# Autodesk Inventor assembly: Assembly1
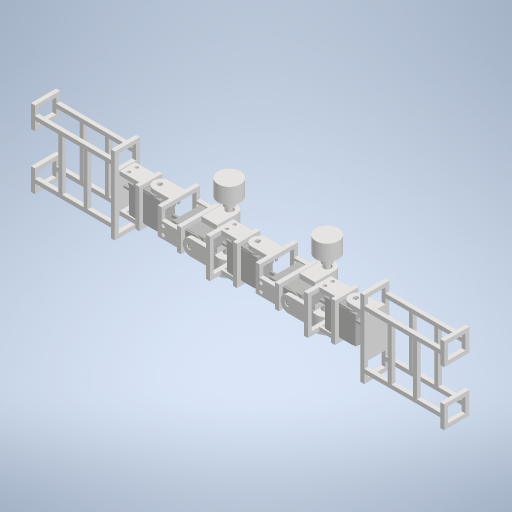
[picture p0: Inventor's stored thumbnail of the model, 512x512]
Saved by Autodesk Inventor 2024 (Build 280153000, 153)
## iProperties
Created: 2023-06-11
Part Number: Assembly1
Document SubType Name: Assembly
Designer: abhin
Author: abhin
## Documents named in this file (8)
- D:\Parth Folder\ES117\3D Model\Prototype 2\MBody(1).iam
- D:\Parth Folder\ES117\3D Model\Prototype 2\MG996R.ipt
- D:\Parth Folder\ES117\3D Model\Prototype 2\Sub Unit.ipt
- D:\Parth Folder\ES117\3D Model\Prototype 2\Wheel Holder.ipt
- D:\Parth Folder\ES117\3D Model\Prototype 2\Axis(1).ipt
- D:\Parth Folder\ES117\3D Model\Prototype 2\Small Wheels.ipt
- D:\Parth Folder\ES117\3D Model\Prototype 2\MHead(1).ipt
- D:\Parth Folder\ES117\3D Model\Prototype 2\MTail(1).ipt
## Components (19 placed, 7 different names)
1. MG996R:1 — Mate:1, Mate:2, Flush:1, Mate:31, Mate:32
2. Sub Unit:1 — Mate:1, Mate:2, Flush:1, Mate:3, Mate:4
3. MG996R:2 — Mate:3, Mate:4, Mate:5, Mate:6, Flush:2, Mate:19, Mate:20, Flush:6
4. Sub Unit:2 — Mate:5, Mate:6, Flush:2, Mate:9, Mate:10
5. MG996R:3 — Mate:9, Mate:10
6. Sub Unit:3 — Mate:13, Mate:14
7. MG996R:4 — Mate:13, Mate:14, Mate:17, Mate:18, Flush:5
8. Sub Unit:4 — Mate:15, Mate:16
9. MG996R:5 — Mate:15, Mate:16, Flush:9, Mate:33, Mate:34
10. Wheel Holder:1 — Mate:17, Mate:18, Flush:5, Mate:21, Flush:7
11. Wheel Holder:2 — Mate:19, Mate:20, Flush:6, Mate:22, Flush:8
12. Axis(1):1 — Mate:21, Flush:7, Mate:23, Mate:26, Mate:27, Mate:30
13. Axis(1):2 — Mate:22, Flush:8, Mate:24, Mate:25, Mate:28, Mate:29
14. Small Wheels:1 — Mate:26, Mate:30
15. Small Wheels:2 — Mate:25, Mate:29
16. Small Wheels:3 — Mate:23, Mate:27
17. Small Wheels:4 — Mate:24, Mate:28
18. MHead(1):1 — Mate:31, Mate:32
19. MTail(1):1 — Flush:9, Mate:33, Mate:34
## Relationships (43: Mate 34, Flush 9)
- Mate:1: MG996R:1 ↔ Sub Unit:1
- Mate:2: MG996R:1 ↔ Sub Unit:1
- Flush:1: MG996R:1 ↔ Sub Unit:1
- Mate:3: Sub Unit:1 ↔ MG996R:2
- Mate:4: Sub Unit:1 ↔ MG996R:2
- Mate:5: MG996R:2 ↔ Sub Unit:2
- Mate:6: MG996R:2 ↔ Sub Unit:2
- Flush:2: MG996R:2 ↔ Sub Unit:2
- [Mate]: MG996R:3 ↔ Sub Unit:3
- [Mate]: MG996R:3 ↔ Sub Unit:3
- [Flush]: MG996R:3 ↔ Sub Unit:3
- Mate:9: Sub Unit:2 ↔ MG996R:3
- Mate:10: Sub Unit:2 ↔ MG996R:3
- [Mate]: MG996R:4 ↔ Sub Unit:4
- [Mate]: MG996R:4 ↔ Sub Unit:4
- [Flush]: MG996R:4 ↔ Sub Unit:4
- Mate:13: Sub Unit:3 ↔ MG996R:4
- Mate:14: Sub Unit:3 ↔ MG996R:4
- Mate:15: Sub Unit:4 ↔ MG996R:5
- Mate:16: Sub Unit:4 ↔ MG996R:5
- Mate:17: MG996R:4 ↔ Wheel Holder:1
- Mate:18: MG996R:4 ↔ Wheel Holder:1
- Flush:5: MG996R:4 ↔ Wheel Holder:1
- Mate:19: MG996R:2 ↔ Wheel Holder:2
- Mate:20: MG996R:2 ↔ Wheel Holder:2
- Flush:6: MG996R:2 ↔ Wheel Holder:2
- Mate:21: Wheel Holder:1 ↔ Axis(1):1
- Mate:22: Wheel Holder:2 ↔ Axis(1):2
- Flush:7 (30 mm): Wheel Holder:1 ↔ Axis(1):1
- Flush:8 (30 mm): Wheel Holder:2 ↔ Axis(1):2
- Mate:23: Axis(1):1 ↔ Small Wheels:3
- Mate:24: Axis(1):2 ↔ Small Wheels:4
- Mate:25: Axis(1):2 ↔ Small Wheels:2
- Mate:26: Axis(1):1 ↔ Small Wheels:1
- Mate:27: Axis(1):1 ↔ Small Wheels:3
- Mate:28: Axis(1):2 ↔ Small Wheels:4
- Mate:29: Axis(1):2 ↔ Small Wheels:2
- Mate:30: Axis(1):1 ↔ Small Wheels:1
- Mate:31: MG996R:1 ↔ MHead(1):1
- Mate:32: MG996R:1 ↔ MHead(1):1
- Flush:9: MG996R:5 ↔ MTail(1):1
- Mate:33: MG996R:5 ↔ MTail(1):1
- Mate:34: MG996R:5 ↔ MTail(1):1
## Named parameters: d9_d0 = 0 mm, d10_d1 = 0 mm, d11_d2 = 0 mm, d14_d6 = 0 mm, d15_d7 = 0 mm, d16_d8 = 0 mm
